# Autodesk Inventor assembly: 620-1
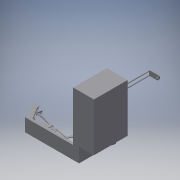
[picture p0: Inventor's stored thumbnail of the model, 180x180]
Saved by Autodesk Inventor 2017 (Build 210142000, 142)
## iProperties
Part Number: 620-1
Material: 一般
Document SubType Name: Assembly
Designer: user
Author: user
## Documents named in this file (14)
- C:\Users\user\Desktop\620\620-1.iam
- C:\Users\user\Desktop\新增資料夾\底座.ipt
- C:\Users\user\Desktop\新增資料夾\軸2mm.ipt
- C:\Users\user\Desktop\新增資料夾\圓盤.ipt
- C:\Users\user\Desktop\新增資料夾\軸4mm.ipt
- C:\Users\user\Desktop\新增資料夾\三角塊3.ipt
- C:\Users\user\Desktop\新增資料夾\連桿4.ipt
- C:\Users\user\Desktop\新增資料夾\三角塊4.ipt
- C:\Users\user\Desktop\新增資料夾\連桿3.ipt
- C:\Users\user\Desktop\新增資料夾\三角塊2.ipt
- C:\Users\user\Desktop\新增資料夾\連桿2.ipt
- C:\Users\user\Desktop\新增資料夾\三角塊1.ipt
- C:\Users\user\Desktop\新增資料夾\連桿1.ipt
- C:\Users\user\Desktop\620\底座.ipt
## Components (23 placed, 12 different names)
1. 底座:1 — 貼合:1, 齊平:1, 旋轉:1, 旋轉:5, 旋轉:11, 旋轉:16, 旋轉:22, 齊平:4, 貼合:2, 齊平:5, 齊平:6
2. 軸2mm:1 — 旋轉:7, 旋轉:8
3. 軸2mm:2 — 旋轉:1, 旋轉:2
4. 軸2mm:3 — 旋轉:16, 旋轉:17
5. 軸2mm:4 — 旋轉:18, 旋轉:19
6. 軸2mm:5 — 旋轉:13, 旋轉:14
7. 軸2mm:6 — 旋轉:11, 旋轉:12
8. 軸2mm:8 — 旋轉:5, 旋轉:6
9. 軸2mm:9 — 旋轉:9, 旋轉:10
10. 圓盤:1 — 旋轉:2, 旋轉:3, 旋轉:4
11. 軸4mm:1 — 旋轉:3, 旋轉:15
12. 三角塊3:1 — 旋轉:4, 旋轉:8, 旋轉:9
13. 連桿4:1 — 旋轉:6, 旋轉:7
14. 三角塊4:1 — 旋轉:10, 旋轉:14
15. 連桿3:1 — 旋轉:12, 旋轉:13
16. 三角塊2:1 — 旋轉:15, 旋轉:19, 旋轉:20
17. 連桿2:1 — 旋轉:17, 旋轉:18
18. 軸2mm:10 — 旋轉:20, 旋轉:21
19. 軸2mm:11 — 旋轉:22, 旋轉:23
20. 軸2mm:13 — 旋轉:24, 旋轉:25
21. 三角塊1:1 — 旋轉:21, 旋轉:25
22. 連桿1:1 — 旋轉:23, 旋轉:24
23. 底座:2 — 貼合:2, 齊平:5, 齊平:6
## Relationships (31: RevoluteJoint 25, Flush 4, Mate 2)
- 貼合:1 [Mate]: 底座:1
- 齊平:1 [Flush]: 底座:1
- 旋轉:1 [RevoluteJoint]: 底座:1 ↔ 軸2mm:2
- 旋轉:2 [RevoluteJoint]: 軸2mm:2 ↔ 圓盤:1
- 旋轉:3 [RevoluteJoint]: 圓盤:1 ↔ 軸4mm:1
- 旋轉:4 [RevoluteJoint]: 圓盤:1 ↔ 三角塊3:1
- 旋轉:5 [RevoluteJoint]: 底座:1 ↔ 軸2mm:8
- 旋轉:6 [RevoluteJoint]: 軸2mm:8 ↔ 連桿4:1
- 旋轉:7 [RevoluteJoint]: 軸2mm:1 ↔ 連桿4:1
- 旋轉:8 [RevoluteJoint]: 軸2mm:1 ↔ 三角塊3:1
- 旋轉:9 [RevoluteJoint]: 軸2mm:9 ↔ 三角塊3:1
- 旋轉:10 [RevoluteJoint]: 軸2mm:9 ↔ 三角塊4:1
- 旋轉:11 [RevoluteJoint]: 底座:1 ↔ 軸2mm:6
- 旋轉:12 [RevoluteJoint]: 軸2mm:6 ↔ 連桿3:1
- 旋轉:13 [RevoluteJoint]: 軸2mm:5 ↔ 連桿3:1
- 旋轉:14 [RevoluteJoint]: 軸2mm:5 ↔ 三角塊4:1
- 旋轉:15 [RevoluteJoint]: 軸4mm:1 ↔ 三角塊2:1
- 旋轉:16 [RevoluteJoint]: 底座:1 ↔ 軸2mm:3
- 旋轉:17 [RevoluteJoint]: 軸2mm:3 ↔ 連桿2:1
- 旋轉:18 [RevoluteJoint]: 軸2mm:4 ↔ 連桿2:1
- 旋轉:19 [RevoluteJoint]: 軸2mm:4 ↔ 三角塊2:1
- 旋轉:20 [RevoluteJoint]: 三角塊2:1 ↔ 軸2mm:10
- 旋轉:21 [RevoluteJoint]: 軸2mm:10 ↔ 三角塊1:1
- 旋轉:22 [RevoluteJoint]: 底座:1 ↔ 軸2mm:11
- 旋轉:23 [RevoluteJoint]: 軸2mm:11 ↔ 連桿1:1
- 旋轉:24 [RevoluteJoint]: 軸2mm:13 ↔ 連桿1:1
- 旋轉:25 [RevoluteJoint]: 軸2mm:13 ↔ 三角塊1:1
- 齊平:4 [Flush]: 底座:1
- 貼合:2 [Mate]: 底座:1 ↔ 底座:2
- 齊平:5 [Flush]: 底座:1 ↔ 底座:2
- 齊平:6 [Flush]: 底座:1 ↔ 底座:2
